# Autodesk Inventor assembly: PowellLNR25M
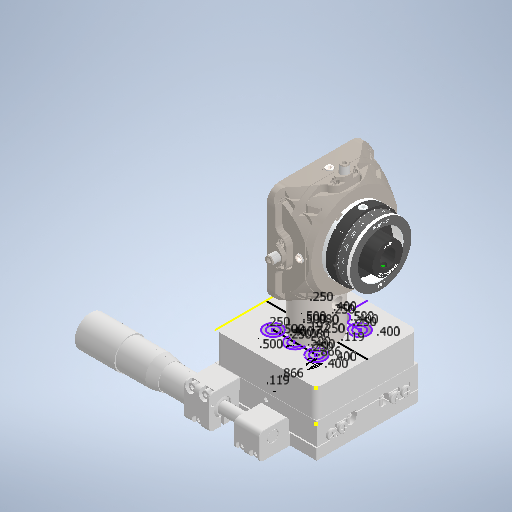
[picture p0: Inventor's stored thumbnail of the model, 512x512]
Saved by Autodesk Inventor 2025.2 (Build 292293000, 293)
## iProperties
Created: 2026-01-29
Part Number: PowellLNR25M
Document SubType Name: Assembly
Designer: monolithic
Author: monolithic
## Documents named in this file (5)
- C:\Users\monolithic\Documents\GitHub\CAD\Monolith\John\Altair_PowellAndCylindricalBaseplatesCombined_10_16_2025\Assemblies\Subassemblies\PowellLNR25M.iam
- C:\Users\monolithic\Documents\GitHub\CAD\Monolith\John\Altair_PowellAndCylindricalBaseplatesCombined_10_16_2025\Assemblies\Subassemblies\LNR25M-Step.ipt
- C:\Users\monolithic\Documents\GitHub\CAD\Monolith\John\LNR25MtoPolarisAdapter\LNR25MtoPolarisAdapter.ipt
- C:\Users\monolithic\Documents\GitHub\CAD\Monolith\John\Altair_PowellAndCylindricalBaseplatesCombined_10_16_2025\Assemblies\Subassemblies\PLS-P1.ipt
- C:\Users\monolithic\Documents\GitHub\CAD\Monolith\John\Altair_PowellAndCylindricalBaseplatesCombined_10_16_2025\Assemblies\Subassemblies\Powell_justXYAssembly.iam
## Components (4 placed, 4 different names)
1. LNR25M-Step:1 — Mate:4
2. LNR25MtoPolarisAdapter:1 — Mate:2, Mate:3, Mate:4, Angle:1
3. PLS-P1:1 — Mate:2, Mate:3, Mate:5, Mate:6
4. Powell_justXYAssembly:1 [sub-assembly] — Mate:5, Mate:6, Angle:1
## Relationships (6: Mate 5, Angle 1)
- Mate:2: LNR25MtoPolarisAdapter:1 ↔ PLS-P1:1
- Mate:3: LNR25MtoPolarisAdapter:1 ↔ PLS-P1:1
- Mate:4: LNR25M-Step:1 ↔ LNR25MtoPolarisAdapter:1
- Mate:5: PLS-P1:1 ↔ Powell_justXYAssembly:1
- Mate:6: PLS-P1:1 ↔ Powell_justXYAssembly:1
- Angle:1 (180 deg): LNR25MtoPolarisAdapter:1 ↔ Powell_justXYAssembly:1
